# Autodesk Inventor assembly: Поворотный_модуль
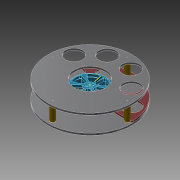
[picture p0: Inventor's stored thumbnail of the model, 180x180]
Saved by Autodesk Inventor 2022 (Build 260153000, 153)
## iProperties
Part Number: Поворотный_модуль
Checked By: Якушев
Engr Approved By: Малов
Material: Типовые
Document SubType Name: Assembly
Mfg Approved By: Судаков
Designer: Смирнов
Author: Смирнов
## Documents named in this file (6)
- E:\4. Прочее\1517\Предпрофессиональная олимпиада\Shoter_V4\Поворотный_модуль.iam
- E:\4. Прочее\1517\Предпрофессиональная олимпиада\Shoter_V4\Диск_опорный.ipt
- E:\4. Прочее\1517\Предпрофессиональная олимпиада\Shoter_V4\Фиксатор.ipt
- E:\4. Прочее\1517\Предпрофессиональная олимпиада\Shoter_V4\Стойка.ipt
- E:\4. Прочее\1517\Предпрофессиональная олимпиада\Shoter_V4\Диск_фиксирующий.ipt
- E:\4. Прочее\1517\Предпрофессиональная олимпиада\Shoter_V4\Переходник.ipt
## Components (8 placed, 5 different names)
1. Диск_опорный:1 — Заподлицо:1, Совмещение:1, Совмещение:2, Совмещение:3, Совмещение:4
2. Фиксатор:1 — Заподлицо:1
3. Диск_фиксирующий:1 — Заподлицо:2
4. Переходник:1 — Совмещение:3, Совмещение:4
5. Стойка:1 — Совмещение:1, Совмещение:2
6. Стойка:2
7. Стойка:3 — Заподлицо:2
8. Стойка:4
## Component patterns: (4 elements, first: Стойка:1)
## Relationships (6: Mate 4, Flush 2)
- Заподлицо:1 [Flush]: Диск_опорный:1 ↔ Фиксатор:1
- Совмещение:1 [Mate]: Диск_опорный:1 ↔ Стойка:1
- Совмещение:2 [Mate]: Диск_опорный:1 ↔ Стойка:1
- Заподлицо:2 [Flush]: Диск_фиксирующий:1 ↔ Стойка:3
- Совмещение:3 [Mate]: Диск_опорный:1 ↔ Переходник:1
- Совмещение:4 [Mate]: Диск_опорный:1 ↔ Переходник:1
